# Autodesk Inventor assembly: 部件1
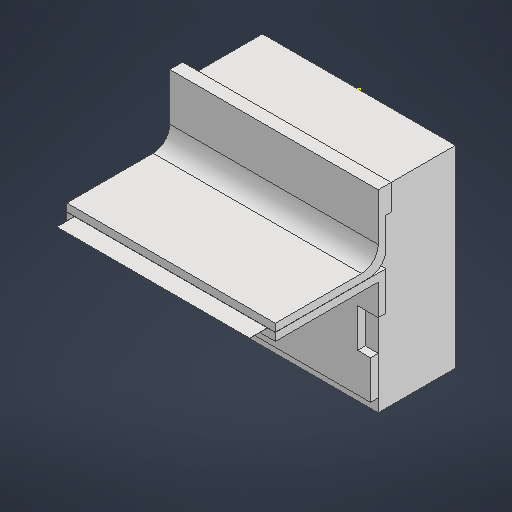
[picture p0: Inventor's stored thumbnail of the model, 512x512]
Saved by Autodesk Inventor 2025 (Build 290162000, 162)
## iProperties
Created: 2025-11-30
Part Number: 部件1
Document SubType Name: Assembly
Designer: XH
Author: XH
## Documents named in this file (4)
- D:\2 B Mechanical design\braille-printer-v2\部件1.iam
- D:\2 B Mechanical design\braille-printer-v2\便签.ipt
- D:\2 B Mechanical design\braille-printer-v2\主体.ipt
- D:\2 B Mechanical design\braille-printer-v2\前舵机位置控制.ipt
## Components (3 placed, 3 different names)
1. 便签:1 — 配合:1, 表面齐平:1, 配合:2, 配合:3
2. 主体:1 — 配合:1, 表面齐平:1, 配合:2
3. 前舵机位置控制:1 — 配合:3
## Relationships (4: Mate 3, Flush 1)
- 配合:1 [Mate]: 便签:1 ↔ 主体:1
- 表面齐平:1 [Flush]: 便签:1 ↔ 主体:1
- 配合:2 [Mate]: 便签:1 ↔ 主体:1
- 配合:3 [Mate]: 便签:1 ↔ 前舵机位置控制:1
